# Autodesk Inventor assembly: ExteriorBumperCar
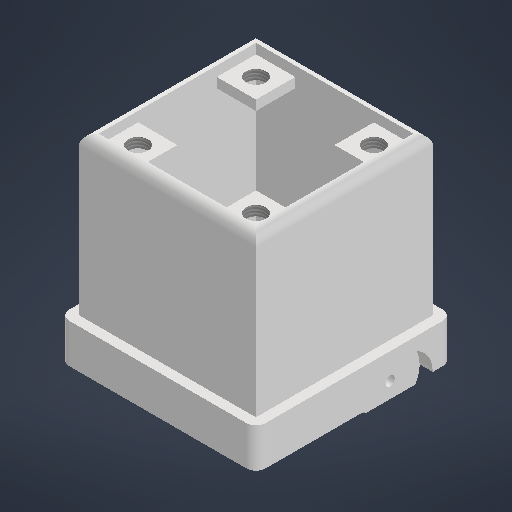
[picture p0: Inventor's stored thumbnail of the model, 512x512]
Saved by Autodesk Inventor 2026.1 (Build 301233000, 233)
## iProperties
Created: 2026-06-28
Part Number: ExteriorBumperCar
Document SubType Name: Assembly
Designer: Kasi Pusuluri
Author: Kasi Pusuluri
## Documents named in this file (7)
- C:\Users\Kasi Pusuluri\Documents\Outpost 2026\BumperCarV2\ExteriorBumperCar.iam
- C:\Users\Kasi Pusuluri\Documents\Outpost 2026\BumperCarV2\BumperBody.ipt
- C:\Users\Kasi Pusuluri\Documents\Outpost 2026\BumperCarV2\Connector1.ipt
- C:\Users\Kasi Pusuluri\Documents\Outpost 2026\BumperCarV2\MotorProtector.ipt
- C:\Users\Kasi Pusuluri\Documents\Outpost 2026\BumperCarV2\Base.ipt
- C:\Users\Kasi Pusuluri\Documents\Outpost 2026\BumperCarV2\WheelConnector.ipt
- C:\Users\Kasi Pusuluri\Documents\Outpost 2026\BumperCarV2\Top.ipt
## Components (11 placed, 6 different names)
1. BumperBody:1 — Rigid:1, Rigid:2, Mate:1, Mate:2, Mate:3, Mate:4
2. Connector1:1 — Rotational:3
3. Connector1:2 — Rotational:2
4. Connector1:3 — Rotational:1
5. Connector1:4 — Rotational:4
6. MotorProtector:1 — Rigid:1
7. MotorProtector:2 — Rigid:2
8. Base:1 — Mate:1, Mate:2
9. WheelConnector:1
10. WheelConnector:2
11. Top:1 — Rotational:1, Rotational:2, Rotational:3, Rotational:4, Mate:3, Mate:4
## Relationships (10: Mate 4, RevoluteJoint 4, WeldJoint 2)
- Rigid:1 [WeldJoint]: BumperBody:1 ↔ MotorProtector:1
- Rigid:2 [WeldJoint]: BumperBody:1 ↔ MotorProtector:2
- Mate:1: BumperBody:1 ↔ Base:1
- Mate:2: BumperBody:1 ↔ Base:1
- Rotational:1 [RevoluteJoint]: Connector1:3 ↔ Top:1
- Rotational:2 [RevoluteJoint]: Connector1:2 ↔ Top:1
- Rotational:3 [RevoluteJoint]: Connector1:1 ↔ Top:1
- Rotational:4 [RevoluteJoint]: Connector1:4 ↔ Top:1
- Mate:3: BumperBody:1 ↔ Top:1
- Mate:4: BumperBody:1 ↔ Top:1
